# Autodesk Inventor assembly: assembly
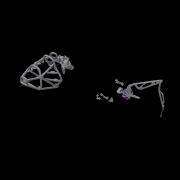
[picture p0: Inventor's stored thumbnail of the model, 180x180]
Saved by Autodesk Inventor 2020 (Build 240168000, 168)
## iProperties
Created: 2020-03-24
Part Number: assembly
Document SubType Name: Assembly
Designer: valer
Author: valer
## Documents named in this file (13)
- C:\Users\valer\Desktop\drummingrobot\src\Robot.iam
- C:\Users\valer\Desktop\drummingrobot\src\Chest.ipt
- C:\Users\valer\Desktop\drummingrobot\src\HeadScaled.ipt
- C:\Users\valer\Desktop\drummingrobot\src\UpperArmServoDynamixelXM430-W350-T.ipt
- C:\Users\valer\Desktop\drummingrobot\src\Forearm.ipt
- C:\Users\valer\Desktop\drummingrobot\src\UpperArm.ipt
- C:\Users\valer\Desktop\drummingrobot\src\UpperArmBracket.ipt
- C:\Users\valer\Desktop\drummingrobot\src\UpperArmMount.ipt
- C:\Users\valer\Desktop\drummingrobot\src\ShoulderBracket.ipt
- C:\Users\valer\Desktop\drummingrobot\src\ShoulderChestBracket.ipt
- C:\Users\valer\Desktop\drummingrobot\src\external\ShoulderConnectingRod.ipt
- C:\Users\valer\Desktop\drummingrobot\src\external\RodEnd.ipt
- C:\Users\valer\Desktop\drummingrobot\src\external\RodEndBall.ipt
## Components (31 placed, 12 different names)
1. Chest:1 — Angle:1, Mate:16, Angle:4
2. HeadScaled:1
3. UpperArmServoDynamixelXM430-W350-T:1 — Angle:1, Mate:10, Mate:11, Mate:12, Mate:13, Mate:14, Angle:2, Mate:15
4. Forearm:1 — Mate:1, Flush:1
5. UpperArm:1 — Mate:1, Flush:1, Mate:2, Mate:3, Mate:4, Mate:5
6. UpperArmBracket:1 — Mate:2, Mate:3, Mate:6, Mate:8, Mate:25
7. UpperArmMount:1 — Mate:6, Mate:7, Mate:8, Mate:10, Mate:11, Angle:3, Angle:5, Mate:25
8. UpperArmBracket:2 — Mate:4, Mate:5, Mate:7
9. ShoulderBracket:1 — Mate:12, Mate:14, Angle:2
10. ShoulderBracket:2 — Mate:13, Mate:15, Angle:3
11. ShoulderChestBracket:1 — Mate:16, Angle:4, Angle:5
12. ChestConnectingRod:1 — Mate:17, Mate:18, Mate:19, Mate:20
13. ChestConnectingRod:2 — Mate:26, Mate:27, Mate:28, Mate:29
14. ChestConnectingRod:3
15. ChestConnectingRod:4 — Mate:34, Mate:35, Mate:36, Mate:37
16. RodEnd:1 — Mate:19, Mate:20, Mate:32
17. RodEnd:2 — Mate:17, Mate:18, Mate:30
18. RodEnd:3 — Mate:26, Mate:27, Mate:31
19. RodEnd:4 — Mate:28, Mate:29, Mate:33
20. RodEndBall:5 — Mate:30
21. RodEndBall:6 — Mate:33
22. RodEndBall:7 — Mate:31
23. RodEndBall:8 — Mate:32
24. RodEnd:5 — Mate:35, Mate:36
25. RodEnd:6
26. RodEnd:7 — Mate:34, Mate:37
27. RodEnd:8
28. RodEndBall:9
29. RodEndBall:10
30. RodEndBall:11
31. RodEndBall:12
## Relationships (38: Mate 32, Angle 5, Flush 1)
- Angle:1 (0 deg): Chest:1 ↔ UpperArmServoDynamixelXM430-W350-T:1
- Mate:1: Forearm:1 ↔ UpperArm:1
- Flush:1 (12.7 mm): Forearm:1 ↔ UpperArm:1
- Mate:2: UpperArm:1 ↔ UpperArmBracket:1
- Mate:3: UpperArm:1 ↔ UpperArmBracket:1
- Mate:4: UpperArm:1 ↔ UpperArmBracket:2
- Mate:5: UpperArm:1 ↔ UpperArmBracket:2
- Mate:6: UpperArmBracket:1 ↔ UpperArmMount:1
- Mate:7: UpperArmMount:1 ↔ UpperArmBracket:2
- Mate:8: UpperArmBracket:1 ↔ UpperArmMount:1
- Mate:10: UpperArmServoDynamixelXM430-W350-T:1 ↔ UpperArmMount:1
- Mate:11: UpperArmServoDynamixelXM430-W350-T:1 ↔ UpperArmMount:1
- Mate:12: UpperArmServoDynamixelXM430-W350-T:1 ↔ ShoulderBracket:1
- Mate:13: UpperArmServoDynamixelXM430-W350-T:1 ↔ ShoulderBracket:2
- Mate:14: UpperArmServoDynamixelXM430-W350-T:1 ↔ ShoulderBracket:1
- Angle:2 (0 deg): UpperArmServoDynamixelXM430-W350-T:1 ↔ ShoulderBracket:1
- Mate:15: UpperArmServoDynamixelXM430-W350-T:1 ↔ ShoulderBracket:2
- Angle:3 (0 deg): UpperArmMount:1 ↔ ShoulderBracket:2
- Mate:16 (6.35 mm): Chest:1 ↔ ShoulderChestBracket:1
- Angle:4 (0 deg): Chest:1 ↔ ShoulderChestBracket:1
- Mate:17: ChestConnectingRod:1 ↔ RodEnd:2
- Mate:18 (-25.4 mm): ChestConnectingRod:1 ↔ RodEnd:2
- Mate:19: ChestConnectingRod:1 ↔ RodEnd:1
- Mate:20 (-25.4 mm): ChestConnectingRod:1 ↔ RodEnd:1
- Angle:5 (0 deg): UpperArmMount:1 ↔ ShoulderChestBracket:1
- Mate:25 (12.7 mm): UpperArmBracket:1 ↔ UpperArmMount:1
- Mate:26: ChestConnectingRod:2 ↔ RodEnd:3
- Mate:27 (-25.4 mm): ChestConnectingRod:2 ↔ RodEnd:3
- Mate:28: ChestConnectingRod:2 ↔ RodEnd:4
- Mate:29 (-25.4 mm): ChestConnectingRod:2 ↔ RodEnd:4
- Mate:30: RodEnd:2 ↔ RodEndBall:5
- Mate:31: RodEnd:3 ↔ RodEndBall:7
- Mate:32: RodEnd:1 ↔ RodEndBall:8
- Mate:33: RodEnd:4 ↔ RodEndBall:6
- Mate:34: ChestConnectingRod:4 ↔ RodEnd:7
- Mate:35: ChestConnectingRod:4 ↔ RodEnd:5
- Mate:36 (-25.4 mm): ChestConnectingRod:4 ↔ RodEnd:5
- Mate:37 (-25.4 mm): ChestConnectingRod:4 ↔ RodEnd:7
